# Autodesk Inventor assembly: C_v2
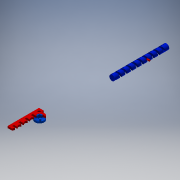
[picture p0: Inventor's stored thumbnail of the model, 180x180]
Saved by Autodesk Inventor 2019 (Build 230136000, 136)
## iProperties
Created: 2020-03-27
Part Number: C_v2
Document SubType Name: Assembly
Designer: Pulag
Author: Pulag
## Documents named in this file (5)
- C:\Users\Pulag\Documents\GitHub\24th_TDK_Project_D5\CAD\frame\日內瓦機構\C_v2.iam
- C:\Users\Pulag\Documents\GitHub\24th_TDK_Project_D5\CAD\frame\A.ipt
- C:\Users\Pulag\Documents\GitHub\24th_TDK_Project_D5\CAD\frame\C.ipt
- C:\Users\Pulag\Documents\GitHub\24th_TDK_Project_D5\CAD\frame\日內瓦機構\rotation.ipt
- C:\Users\Pulag\Documents\GitHub\24th_TDK_Project_D5\CAD\frame\日內瓦機構\rotation 2.ipt
## Components (4 placed, 4 different names)
1. A:1 — Mate:3, Mate:4
2. C:1 — Mate:1, Mate:2, Mate:3
3. rotation:1 — Mate:5, Mate:6, Mate:7
4. rotation 2:1 — Mate:7, Mate:8
## Relationships (8: Mate 8)
- Mate:1: C:1
- Mate:2: C:1
- Mate:3: A:1 ↔ C:1
- Mate:4 (-7.7 mm): A:1
- Mate:5 (80 mm): rotation:1
- Mate:6: rotation:1
- Mate:7 (2 mm): rotation:1 ↔ rotation 2:1
- Mate:8: rotation 2:1
